# Autodesk Inventor assembly: skirtback
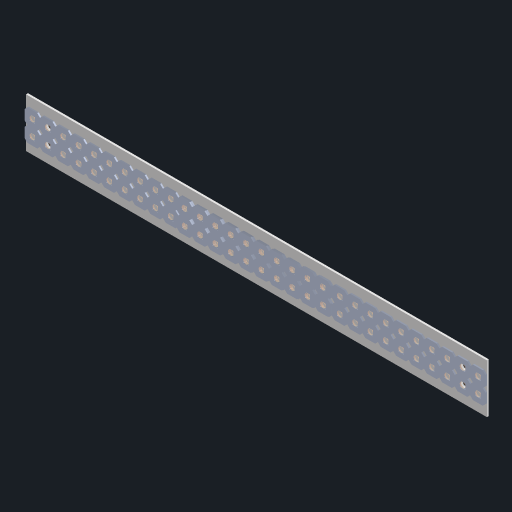
[picture p0: Inventor's stored thumbnail of the model, 512x512]
Saved by Autodesk Inventor 2023 (Build 270158000, 158)
## iProperties
Created: 2023-04-10
Part Number: skirtback
Document SubType Name: Assembly
Designer: Windows Macbook
Author: Windows Macbook
## Documents named in this file (4)
- C:\Users\Windows Macbook\Desktop\VRC-SPIN-UP\Inventor\Assembly\Worlds\skirtback.iam
- C:\Users\Windows Macbook\Desktop\VRC-SPIN-UP\Inventor\Assembly\Worlds\skirtback.ipt
- C:\Users\Windows Macbook\Desktop\VRC-SPIN-UP\Inventor\Structure\Plate\Steel\Steel Plate 2x15.ipt
- C:\Users\Windows Macbook\Desktop\VRC-SPIN-UP\Inventor\Structure\Plate\Steel\Steel Plate 2x10.ipt
## Components (4 placed, 3 different names)
1. skirtback:1 — Insert:1, Insert:2, Insert:3, Insert:4
2. Steel Plate 2x15:2 — Insert:1, Insert:2, Insert:5
3. Steel Plate 2x15:1 — Insert:3, Insert:4
4. Steel Plate 2x10:1 — Insert:5
## Relationships (5: Insert 5)
- Insert:1: skirtback:1 ↔ Steel Plate 2x15:2
- Insert:2: skirtback:1 ↔ Steel Plate 2x15:2
- Insert:3: skirtback:1 ↔ Steel Plate 2x15:1
- Insert:4: skirtback:1 ↔ Steel Plate 2x15:1
- Insert:5: Steel Plate 2x15:2 ↔ Steel Plate 2x10:1
